# Autodesk Inventor assembly: 2024_0210_Wheel_A
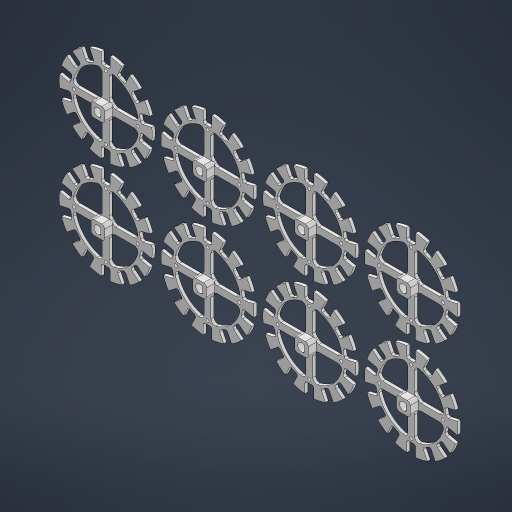
[picture p0: Inventor's stored thumbnail of the model, 512x512]
Saved by Autodesk Inventor 2024.2 (Build 282272000, 272)
## iProperties
Created: 2024-02-10
Part Number: 2024_0210_Wheel_A
Document SubType Name: Assembly
Designer: Hanaoka
Author: Hanaoka
## Documents named in this file (2)
- G:\共有ドライブ\reRo\05_個人\hanaoka\inventor\CAMpath\2024_0210_Wheel_A.iam
- G:\共有ドライブ\reRo\05_個人\hanaoka\inventor\DriveUnit\OmniFrame_A.ipt
## Components (8 placed, 1 different names)
1. OmniFrame_A:1 — メイト:1, メイト:2, 正接:1
2. OmniFrame_A:2
3. OmniFrame_A:3
4. OmniFrame_A:4
5. OmniFrame_A:5
6. OmniFrame_A:6
7. OmniFrame_A:7
8. OmniFrame_A:8
## Component patterns: (8 elements, first: OmniFrame_A:1)
## Relationships (3: Mate 2, Tangent 1)
- メイト:1 [Mate]: OmniFrame_A:1
- メイト:2 [Mate] (6 mm): OmniFrame_A:1
- 正接:1 [Tangent]: OmniFrame_A:1
